# Autodesk Inventor assembly: extruder assembly
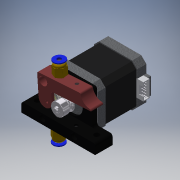
[picture p0: Inventor's stored thumbnail of the model, 180x180]
Saved by Autodesk Inventor 2016 SP1 (Build 200210100, 210)
## iProperties
Created: 2015-12-27
Part Number: extruder assembly
Document SubType Name: Assembly
Designer: Dirk Alferink
Author: Dirk Alferink
## Documents named in this file (7)
- C:\Users\ubik\Dropbox\proiecte\inventor\kossel\extruder assembly.iam
- C:\Users\ubik\Dropbox\proiecte\inventor\kossel\Part1.ipt
- C:\Users\ubik\Dropbox\proiecte\inventor\kossel\Part2.ipt
- C:\Users\ubik\Dropbox\proiecte\inventor\kossel\NEMA17 Stepper.ipt
- C:\Users\ubik\Dropbox\proiecte\inventor\kossel\Bowden.ipt
- C:\Users\ubik\Dropbox\proiecte\inventor\kossel\Drive Gear.ipt
- C:\Users\ubik\Dropbox\proiecte\inventor\kossel\idler bearing.ipt
## Components (7 placed, 6 different names)
1. Part1:1 — Insert:1, Insert:2, Insert:3, Insert:5
2. Part2:1 — Insert:3, Insert:4, Insert:13
3. NEMA17 Stepper:1 — Insert:1, Insert:2, Insert:6
4. Bowden:1 — Insert:4
5. Bowden:2 — Insert:5
6. Drive Gear:1 — Insert:6
7. idler bearing:1 — Insert:13
## Relationships (7: Insert 7)
- Insert:1: Part1:1 ↔ NEMA17 Stepper:1
- Insert:2: Part1:1 ↔ NEMA17 Stepper:1
- Insert:3: Part1:1 ↔ Part2:1
- Insert:4: Part2:1 ↔ Bowden:1
- Insert:5: Part1:1 ↔ Bowden:2
- Insert:6 (1 mm): NEMA17 Stepper:1 ↔ Drive Gear:1
- Insert:13: Part2:1 ↔ idler bearing:1
